# Autodesk Inventor assembly: Assembly_Eyepiece_Folded_longtube
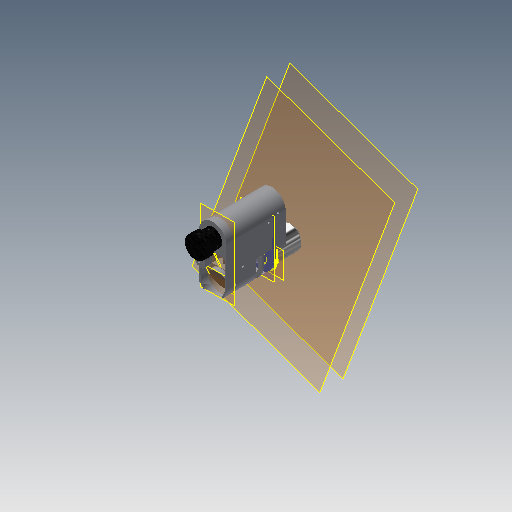
[picture p0: Inventor's stored thumbnail of the model, 512x512]
Saved by Autodesk Inventor 2019 (Build 230136000, 136)
## iProperties
Created: 2019-11-14
Part Number: Assembly_Eyepiece_Folded_longtube
Document SubType Name: Assembly
Designer: diederichbenedict
Author: diederichbenedict
## Documents named in this file (6)
- C:\Users\diederichbenedict\Dropbox\Dokumente\Promotion\PROJECTS\STORMoChip\INVENTOR\Nanoscopy-on-a-cheap\Assembly_Eyepiece_Folded_longtube.iam
- C:\Users\diederichbenedict\Dropbox\Dokumente\Promotion\PROJECTS\STORMoChip\INVENTOR\Nanoscopy-on-a-cheap\00_Eyepiece_20x_WF.ipt
- C:\Users\diederichbenedict\Dropbox\Dokumente\Promotion\PROJECTS\STORMoChip\INVENTOR\Nanoscopy-on-a-cheap\00_Microscope_Objective.ipt
- C:\Users\diederichbenedict\Dropbox\Dokumente\Promotion\PROJECTS\STORMoChip\INVENTOR\Nanoscopy-on-a-cheap\PF10-03-P01-Step.ipt
- C:\Users\diederichbenedict\Dropbox\Dokumente\Promotion\PROJECTS\STORMoChip\INVENTOR\Nanoscopy-on-a-cheap\00_Beam_Ocular_Detection_longtube.ipt
- C:\Users\diederichbenedict\Dropbox\Dokumente\Promotion\PROJECTS\STORMoChip\INVENTOR\Nanoscopy-on-a-cheap\cellSTORM_objective_tube_folded_mirror_v0_longtube.ipt
## Components (6 placed, 5 different names)
1. 00_Eyepiece_20x_WF:1 — Insert:5
2. 00_Microscope_Objective:1 — Insert:2, Insert:6
3. PF10-03-P01-Step:1 — Insert:3, Angle:2, Flush:1
4. PF10-03-P01-Step:2 — Insert:4, Angle:3
5. 00_Beam_Ocular_Detection_longtube:1 — Insert:2, Insert:3, Insert:4, Insert:5, Angle:1
6. cellSTORM_objective_tube_folded_mirror_v0_longtube:1 — Insert:6, Angle:1, Angle:2, Angle:3, Flush:1
## Relationships (9: Insert 5, Angle 3, Flush 1)
- Insert:2: 00_Microscope_Objective:1 ↔ 00_Beam_Ocular_Detection_longtube:1
- Insert:3: PF10-03-P01-Step:1 ↔ 00_Beam_Ocular_Detection_longtube:1
- Insert:4: PF10-03-P01-Step:2 ↔ 00_Beam_Ocular_Detection_longtube:1
- Insert:5: 00_Eyepiece_20x_WF:1 ↔ 00_Beam_Ocular_Detection_longtube:1
- Insert:6: 00_Microscope_Objective:1 ↔ cellSTORM_objective_tube_folded_mirror_v0_longtube:1
- Angle:1 (0 deg): 00_Beam_Ocular_Detection_longtube:1 ↔ cellSTORM_objective_tube_folded_mirror_v0_longtube:1
- Angle:2 (90 deg): PF10-03-P01-Step:1 ↔ cellSTORM_objective_tube_folded_mirror_v0_longtube:1
- Angle:3 (90 deg): PF10-03-P01-Step:2 ↔ cellSTORM_objective_tube_folded_mirror_v0_longtube:1
- Flush:1: PF10-03-P01-Step:1 ↔ cellSTORM_objective_tube_folded_mirror_v0_longtube:1
